# Autodesk Inventor assembly: item_0064944_Monitor_Arm_A1=0_A2=0_A3=0_1
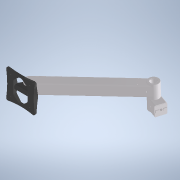
[picture p0: Inventor's stored thumbnail of the model, 180x180]
Saved by Autodesk Inventor 2020 (Build 240168000, 168)
## iProperties
Company: CADClick - www.CADClick.com
Created: 2019-11-06
Part Number: item_0064944_Monitor_Arm_A1=0_A2=0_A3=0_1
Description: STEP AP214
Document SubType Name: Assembly
Designer: nicoc
Authority: unknown authorization
Preprocessor: Spatial InterOp 3D
Title: cctmp_107506AD-F5B5-4EC3-AB72-893FABB32A8D_2019_11_6_15_3_17_13..stp
Author: item Industrietechnik GmbH
Revision Number: NONE
## Documents named in this file (8)
- D:\Repos\P5-AIonFPGA\cad\Display\MonitorHolder\item_0064944_Monitor_Arm_A1=0_A2=0_A3=0_1.iam
- D:\Repos\P5-AIonFPGA\cad\Display\MonitorHolder\item_0064944_Monitor Arm_A1=0_A2=0_A3=0.ipt
- D:\Repos\P5-AIonFPGA\cad\Display\MonitorHolder\item_0064944_Monitor Arm_A1=0_A2=0_A3=0_1.ipt
- D:\Repos\P5-AIonFPGA\cad\Display\MonitorHolder\item_0064944_Monitor Arm_A1=0_A2=0_A3=0_2.ipt
- D:\Repos\P5-AIonFPGA\cad\Display\MonitorHolder\item_0064944_Monitor Arm_A1=0_A2=0_A3=0_9.ipt
- D:\Repos\P5-AIonFPGA\cad\Display\MonitorHolder\item_0064944_Monitor Arm_A1=0_A2=0_A3=0_10.ipt
- D:\Repos\P5-AIonFPGA\cad\Display\MonitorHolder\item_0064944_Monitor Arm_A1=0_A2=0_A3=0_11.ipt
- D:\Repos\P5-AIonFPGA\cad\Display\MonitorHolder\item_0064944_Monitor Arm_A1=0_A2=0_A3=0_12.ipt
## Components (7 placed, 7 different names)
1. item_0064944_Monitor Arm_A1=0_A2=0_A3=0 — Mate:1, Mate:2
2. item_0064944_Monitor Arm_A1=0_A2=0_A3=0_1 — Mate:1, Mate:2, Mate:10, Mate:11
3. item_0064944_Monitor Arm_A1=0_A2=0_A3=0_2 — Mate:4, Flush:1, Flush:2, Mate:10, Mate:11
4. item_0064944_Monitor Arm_A1=0_A2=0_A3=0_9 — Mate:4, Flush:1, Flush:2, Mate:5, Flush:3, Flush:4
5. item_0064944_Monitor Arm_A1=0_A2=0_A3=0_10 — Mate:5, Flush:3, Flush:4, Mate:6, Mate:7, Mate:9
6. item_0064944_Monitor Arm_A1=0_A2=0_A3=0_11 — Mate:8, Mate:9
7. item_0064944_Monitor Arm_A1=0_A2=0_A3=0_12 — Mate:6, Mate:7, Mate:8
## Relationships (14: Mate 10, Flush 4)
- Mate:1 (2.5 mm): item_0064944_Monitor Arm_A1=0_A2=0_A3=0 ↔ item_0064944_Monitor Arm_A1=0_A2=0_A3=0_1
- Mate:2: item_0064944_Monitor Arm_A1=0_A2=0_A3=0 ↔ item_0064944_Monitor Arm_A1=0_A2=0_A3=0_1
- Mate:4: item_0064944_Monitor Arm_A1=0_A2=0_A3=0_2 ↔ item_0064944_Monitor Arm_A1=0_A2=0_A3=0_9
- Flush:1: item_0064944_Monitor Arm_A1=0_A2=0_A3=0_2 ↔ item_0064944_Monitor Arm_A1=0_A2=0_A3=0_9
- Flush:2: item_0064944_Monitor Arm_A1=0_A2=0_A3=0_2 ↔ item_0064944_Monitor Arm_A1=0_A2=0_A3=0_9
- Mate:5: item_0064944_Monitor Arm_A1=0_A2=0_A3=0_9 ↔ item_0064944_Monitor Arm_A1=0_A2=0_A3=0_10
- Flush:3: item_0064944_Monitor Arm_A1=0_A2=0_A3=0_9 ↔ item_0064944_Monitor Arm_A1=0_A2=0_A3=0_10
- Flush:4: item_0064944_Monitor Arm_A1=0_A2=0_A3=0_9 ↔ item_0064944_Monitor Arm_A1=0_A2=0_A3=0_10
- Mate:6: item_0064944_Monitor Arm_A1=0_A2=0_A3=0_10 ↔ item_0064944_Monitor Arm_A1=0_A2=0_A3=0_12
- Mate:7: item_0064944_Monitor Arm_A1=0_A2=0_A3=0_10 ↔ item_0064944_Monitor Arm_A1=0_A2=0_A3=0_12
- Mate:8: item_0064944_Monitor Arm_A1=0_A2=0_A3=0_11 ↔ item_0064944_Monitor Arm_A1=0_A2=0_A3=0_12
- Mate:9: item_0064944_Monitor Arm_A1=0_A2=0_A3=0_10 ↔ item_0064944_Monitor Arm_A1=0_A2=0_A3=0_11
- Mate:10: item_0064944_Monitor Arm_A1=0_A2=0_A3=0_1 ↔ item_0064944_Monitor Arm_A1=0_A2=0_A3=0_2
- Mate:11: item_0064944_Monitor Arm_A1=0_A2=0_A3=0_1 ↔ item_0064944_Monitor Arm_A1=0_A2=0_A3=0_2
